# Autodesk Inventor assembly: 2.75 Traction, Circle_MIR
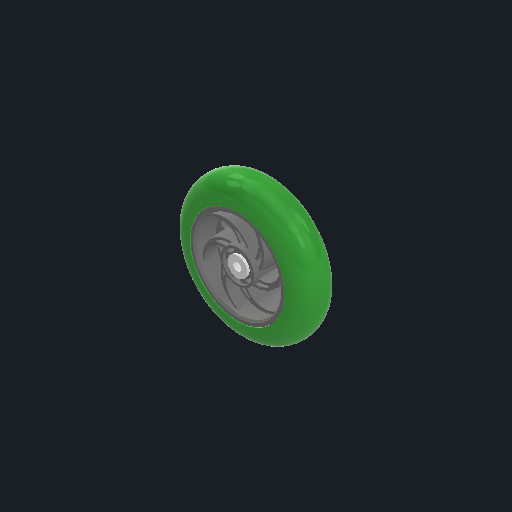
[picture p0: Inventor's stored thumbnail of the model, 512x512]
Saved by Autodesk Inventor 2024 (Build 280153000, 153)
## iProperties
Created: 2022-08-02
Part Number: 2.75 Traction, Circle_MIR
Document SubType Name: Assembly
Designer: macbook
Author: ylu12
## Documents named in this file (3)
- \\Mac\Home\Desktop\code\7899V-VRC-OVER-UNDER\Cad\VEX-CAD-Inventor-1.4.0\Motion\Wheels\Traction Wheel\2.75 Traction, Circle_MIR.iam
- \\Mac\Home\Desktop\code\7899V-VRC-OVER-UNDER\Cad\VEX-CAD-Inventor-1.4.0\Motion\Wheels\Reference Files\2.75 Traction_MIR.ipt
- \\Mac\Home\Desktop\code\7899V-VRC-OVER-UNDER\Cad\VEX-CAD-Inventor-1.4.0\Motion\Insert Circle_MIR.ipt
## Components (3 placed, 2 different names)
1. 2.75 Traction_MIR:1 — Flush:3, Mate:6, Mate:5
2. Insert Circle_MIR:1 — Angle:4, Mate:29, Symmetry:2
3. Insert Circle_MIR:2 — Symmetry:2, Angle:3, Mate:26, Flush:11
## Relationships (9: Mate 5, Angle 2, Flush 1, Symmetry 1)
- Flush:3: 2.75 Traction_MIR:1
- Mate:6: 2.75 Traction_MIR:1
- Mate:5: 2.75 Traction_MIR:1
- Angle:4 (0 deg): Insert Circle_MIR:1
- Mate:29: Insert Circle_MIR:1
- Symmetry:2: Insert Circle_MIR:1 ↔ Insert Circle_MIR:2
- Angle:3 (0 deg): Insert Circle_MIR:2
- Mate:26: Insert Circle_MIR:2
- Flush:11 [Mate] (8.255 mm): Insert Circle_MIR:2
## Named parameters: Thickness = 8.255 mm
